# Autodesk Inventor assembly: Shelf
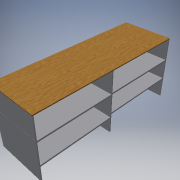
[picture p0: Inventor's stored thumbnail of the model, 180x180]
Saved by Autodesk Inventor 2016 (Build 200138000, 138)
## iProperties
Created: 2016-01-22
Part Number: Shelf
Document SubType Name: Assembly
Designer: yash
Author: yash
## Documents named in this file (4)
- C:\Users\yash\Documents\MakerSpace\MakerSpace\Shelf.iam
- C:\Users\yash\Documents\MakerSpace\MakerSpace\SideDividerWalls.ipt
- C:\Users\yash\Documents\MakerSpace\MakerSpace\TopWood.ipt
- C:\Users\yash\Documents\MakerSpace\MakerSpace\Shelf.ipt
## Components (8 placed, 3 different names)
1. SideDividerWalls:1 — Mate:7, Mate:8, Mate:9, Mate:10, Mate:11, Flush:1, Mate:14, Mate:16
2. TopWood:1 — Mate:1, Mate:2, Mate:3, Mate:4, Mate:5, Mate:6, Mate:7, Mate:9
3. SideDividerWalls:2 — Mate:4, Mate:5, Mate:6, Mate:8, Mate:12
4. SideDividerWalls:3 — Mate:1, Mate:2, Mate:3, Mate:13, Mate:15
5. Shelf:1 — Mate:10, Mate:11
6. Shelf:2 — Mate:12, Flush:1
7. Shelf:3 — Mate:15, Mate:16
8. Shelf:4 — Mate:13, Mate:14
## Relationships (17: Mate 16, Flush 1)
- Mate:1: TopWood:1 ↔ SideDividerWalls:3
- Mate:2: TopWood:1 ↔ SideDividerWalls:3
- Mate:3: TopWood:1 ↔ SideDividerWalls:3
- Mate:4: TopWood:1 ↔ SideDividerWalls:2
- Mate:5: TopWood:1 ↔ SideDividerWalls:2
- Mate:6: TopWood:1 ↔ SideDividerWalls:2
- Mate:7: SideDividerWalls:1 ↔ TopWood:1
- Mate:8 (889 mm): SideDividerWalls:1 ↔ SideDividerWalls:2
- Mate:9: SideDividerWalls:1 ↔ TopWood:1
- Mate:10: SideDividerWalls:1 ↔ Shelf:1
- Mate:11: SideDividerWalls:1 ↔ Shelf:1
- Mate:12: SideDividerWalls:2 ↔ Shelf:2
- Flush:1: SideDividerWalls:1 ↔ Shelf:2
- Mate:13: SideDividerWalls:3 ↔ Shelf:4
- Mate:14: SideDividerWalls:1 ↔ Shelf:4
- Mate:15: SideDividerWalls:3 ↔ Shelf:3
- Mate:16: SideDividerWalls:1 ↔ Shelf:3
